# Autodesk Inventor assembly: Moteur
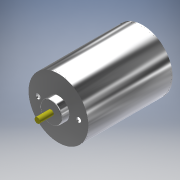
[picture p0: Inventor's stored thumbnail of the model, 180x180]
Saved by Autodesk Inventor 2018 (Build 220112000, 112)
## iProperties
Created: 2017-10-08
Part Number: Moteur
Document SubType Name: Assembly
Designer: liamg
Author: liamg
## Documents named in this file (5)
- C:\Users\liamg\Desktop\Banc_Test_Rotor\Moteur.iam
- C:\Users\liamg\Desktop\Banc_Test_Rotor\Moteur electrique.ipt
- C:\Users\liamg\Desktop\Banc_Test_Rotor\capot_inf.ipt
- C:\Users\liamg\Desktop\Banc_Test_Rotor\capot inférieur.ipt
- C:\Users\liamg\Desktop\Banc_Test_Rotor\Tige d'entraintenement.ipt
## Components (4 placed, 4 different names)
1. Moteur electrique_cylindre:1 — Insert:1, Insert:2
2. Capot superieur — Rotational:1, Insert:1
3. capot inférieur:1 — Insert:2
4. Tige d'entraintenement:1 — Rotational:1
## Relationships (3: Insert 2, RevoluteJoint 1)
- Rotational:1 [RevoluteJoint]: Capot superieur ↔ Tige d'entraintenement:1
- Insert:1: Moteur electrique_cylindre:1 ↔ Capot superieur
- Insert:2: Moteur electrique_cylindre:1 ↔ capot inférieur:1
